# Autodesk Inventor assembly: Assembly.
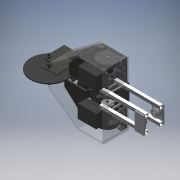
[picture p0: Inventor's stored thumbnail of the model, 180x180]
Saved by Autodesk Inventor 2019 (Build 230136000, 136)
## iProperties
Created: 2018-08-16
Part Number: Assembly.
Document SubType Name: Assembly
Designer: andres2416
Author: andres2416
## Documents named in this file (28)
- O:\Engineering Club Student\Rahul\2018-2019 bot #3\all files\Assembly..iam
- O:\Engineering Club Student\Rahul\2018-2019 bot #3\all files\battery.ipt
- O:\Engineering Club Student\Rahul\2018-2019 bot #3\all files\REAL MOTOR MOUNT 2.75 BOTTOM.ipt
- O:\Engineering Club Student\Rahul\2018-2019 bot #3\all files\REAL MOTOR MOUNT 2.75 TOP.ipt
- O:\Engineering Club Student\Rahul\2018-2019 bot #3\all files\motor.ipt
- O:\Engineering Club Student\Rahul\2018-2019 bot #3\all files\bar for front weapon.ipt
- O:\Engineering Club Student\Rahul\2018-2019 bot #3\all files\standoff.ipt
- O:\Engineering Club Student\Rahul\2018-2019 bot #3\all files\saw blade poly no hole mount.ipt
- O:\Engineering Club Student\Rahul\2018-2019 bot #3\all files\saw blade axle support (hole for arbor).ipt
- O:\Engineering Club Student\Rahul\2018-2019 bot #3\all files\polycarb wall for saw blade.ipt
- O:\Engineering Club Student\Rahul\2018-2019 bot #3\all files\saw blade.ipt
- O:\Engineering Club Student\Rahul\2018-2019 bot #3\all files\6 inch wheel.ipt
- O:\Engineering Club Student\Rahul\2018-2019 bot #3\all files\axle for saw blade.ipt
- O:\Engineering Club Student\Rahul\2018-2019 bot #3\all files\E30-400 motor.ipt
- O:\Engineering Club Student\Rahul\2018-2019 bot #3\all files\MOTOR MOUNT REAL BOTTOM E30 MOTOR.ipt
- O:\Engineering Club Student\Rahul\2018-2019 bot #3\all files\MOTOR MOUNT REAL TOP E3O MOTOR.ipt
- O:\Engineering Club Student\Rahul\2018-2019 bot #3\all files\Very real base.ipt
- O:\Engineering Club Student\Rahul\2018-2019 bot #3\all files\motor mount platform.ipt
- O:\Engineering Club Student\Rahul\2018-2019 bot #3\all files\vex gear.ipt
- O:\Engineering Club Student\Rahul\2018-2019 bot #3\all files\shaft collar for saw blade axle.ipt
- O:\Engineering Club Student\Rahul\2018-2019 bot #3\all files\motor mount platform right side.ipt
- O:\Engineering Club Student\Rahul\2018-2019 bot #3\all files\Front wall.ipt
- O:\Engineering Club Student\Rahul\2018-2019 bot #3\all files\Side wall.ipt
- O:\Engineering Club Student\Rahul\2018-2019 bot #3\all files\rear angled wall.ipt
- O:\Engineering Club Student\Rahul\2018-2019 bot #3\all files\Aluminum Bracket.ipt
- O:\Engineering Club Student\Rahul\2018-2019 bot #3\all files\weapon motor inverted mount.ipt
- O:\Engineering Club Student\Rahul\2018-2019 bot #3\all files\pillowblock].ipt
- O:\Engineering Club Student\Rahul\2018-2019 bot #3\all files\revised pillow block mount.ipt
## Components (59 placed, 27 different names)
1. battery:1 — Mate:10, Flush:20, Flush:21
2. REAL MOTOR MOUNT 2.75 BOTTOM:1 — Insert:8, Insert:39, Insert:40, Flush:15
3. REAL MOTOR MOUNT 2.75 BOTTOM:2 — Insert:37, Insert:38
4. REAL MOTOR MOUNT 2.75 TOP:2 — Insert:11, Insert:12
5. REAL MOTOR MOUNT 2.75 BOTTOM:3 — Insert:11, Insert:12, Insert:31, Insert:32
6. REAL MOTOR MOUNT 2.75 TOP:3 — Insert:13, Insert:14, Mate:1, Flush:39, Flush:40
7. REAL MOTOR MOUNT 2.75 BOTTOM:4 — Insert:7, Insert:13, Insert:14, Insert:29, Insert:30
8. motor:1 — Insert:8, Insert:42, Insert:51
9. motor:2 — Insert:7, Insert:41
10. saw blade poly no hole mount:1 — Mate:14, Flush:27, Flush:28
11. saw blade axle support (hole for arbor):1 — Mate:3, Flush:6, Insert:43
12. polycarb wall for saw blade:1 — Mate:4, Flush:7, Flush:8, Insert:45, Insert:46
13. saw blade:1 — Insert:43, Insert:44
14. 6 inch wheel:1 — Insert:42, Rotation:3
15. 6 inch wheel:2 — Insert:41, Rotation:3
16. axle for saw blade:1 — Insert:44, Insert:47
17. E30-400 motor:1 — Insert:48, Tangent:50, Insert:50, Insert:55
18. MOTOR MOUNT REAL BOTTOM E30 MOTOR:1 — Mate:6, Flush:11, Flush:12, Mate:8, Flush:14
19. MOTOR MOUNT REAL TOP E3O MOTOR:1 — Mate:8, Insert:50, Flush:14
20. MOTOR MOUNT REAL BOTTOM E30 MOTOR:2 — Mate:5, Flush:9, Flush:10, Flush:12, Insert:48, Mate:7, Flush:13
21. MOTOR MOUNT REAL TOP E3O MOTOR:2 — Mate:7, Tangent:50, Flush:13
22. Very real base:1 — Insert:29, Insert:30, Insert:31, Insert:32, Insert:37, Insert:38, Insert:39, Insert:40, Flush:3, Mate:3, Flush:6, Mate:4, Flush:7, Flush:8, Mate:5, Flush:9, Flush:10, Mate:6, Flush:11, Mate:14, Flush:27, Flush:28, Mate:16, Flush:31, Mate:20, Flush:33, Mate:22, Flush:34, Insert:56, Insert:57, Insert:58, Insert:59, Mate:28, Flush:36, Insert:60, Insert:61, Insert:62, Insert:63, Mate:33, Flush:37, Insert:64, Insert:65, Insert:66, Insert:67, Insert:68, Insert:69, Insert:70, Insert:71
23. motor mount platform:1 — Mate:1, Mate:10, Flush:20, Flush:21, Flush:39, Flush:40
24. vex gear:1 — Insert:47
25. vex gear:2 — Insert:55
26. shaft collar for saw blade axle:1 — Insert:45
27. shaft collar for saw blade axle:2 — Insert:46
28. battery:3 — Mate:11, Flush:22
29. REAL MOTOR MOUNT 2.75 TOP:5 — Insert:51, Flush:15, Insert:52, Mate:9, Flush:41
30. REAL MOTOR MOUNT 2.75 TOP:6 — Insert:52, Flush:19
31. motor mount platform right side:1 — Mate:9, Flush:19, Mate:11, Flush:22, Flush:41
32. Side wall:1 — Mate:16, Flush:31, Mate:21, Flush:35, Mate:31, Mate:32
33. rear angled wall:1 — Mate:22, Flush:34, Mate:24, Mate:27
34. rear angled wall:2 — Mate:20, Flush:33, Mate:21, Mate:25, Mate:26
35. Aluminum Bracket:1 — Insert:56, Mate:24
36. Aluminum Bracket:2 — Insert:57, Mate:27
37. Aluminum Bracket:3 — Insert:58, Mate:25
38. Aluminum Bracket:4 — Insert:59, Mate:26
39. Front wall:1 — Mate:28, Flush:35, Flush:36, Mate:29, Mate:30, Mate:34
40. Aluminum Bracket:5 — Insert:61, Mate:30
41. Aluminum Bracket:6 — Insert:60, Mate:29
42. Aluminum Bracket:7 — Insert:65, Mate:36
43. Aluminum Bracket:8 — Insert:64, Mate:35
44. Aluminum Bracket:9 — Insert:63, Mate:32
45. Aluminum Bracket:10 — Insert:62, Mate:31
46. Side wall:2 — Mate:33, Mate:34, Flush:37, Mate:35, Mate:36
47. weapon motor inverted mount:1 — Insert:66, Insert:67
48. pillowblock]:2 — Mate:39, Mate:40, Flush:46
49. bar for front weapon:1 — Insert:78, Insert:79, Mate:38, Flush:44, Flush:45
50. bar for front weapon:2 — Insert:76, Insert:77, Mate:42
51. bar for front weapon:3 — Insert:70, Insert:71, Insert:74, Insert:75, Mate:37, Flush:42, Flush:43
52. bar for front weapon:4 — Insert:68, Insert:69, Insert:72, Insert:73, Mate:40
53. standoff:1 — Insert:75, Insert:78
54. standoff:2 — Insert:74, Insert:79
55. standoff:3 — Insert:73, Insert:76
56. standoff:4 — Insert:72, Insert:77
57. revised pillow block mount:1 — Mate:38, Flush:44, Flush:45, Mate:41, Flush:47
58. revised pillow block mount:2 — Mate:37, Flush:42, Flush:43, Mate:39, Flush:46
59. pillowblock]:3 — Mate:41, Flush:47, Mate:42
## Relationships (118: Insert 50, Mate 34, Flush 32, Tangent 1, RelateRotation 1)
- Insert:7 (-12.7 mm): REAL MOTOR MOUNT 2.75 BOTTOM:4 ↔ motor:2
- Insert:8 (-12.7 mm): REAL MOTOR MOUNT 2.75 BOTTOM:1 ↔ motor:1
- Insert:11: REAL MOTOR MOUNT 2.75 TOP:2 ↔ REAL MOTOR MOUNT 2.75 BOTTOM:3
- Insert:12: REAL MOTOR MOUNT 2.75 TOP:2 ↔ REAL MOTOR MOUNT 2.75 BOTTOM:3
- Insert:13: REAL MOTOR MOUNT 2.75 TOP:3 ↔ REAL MOTOR MOUNT 2.75 BOTTOM:4
- Insert:14: REAL MOTOR MOUNT 2.75 TOP:3 ↔ REAL MOTOR MOUNT 2.75 BOTTOM:4
- Insert:29: REAL MOTOR MOUNT 2.75 BOTTOM:4 ↔ Very real base:1
- Insert:30: REAL MOTOR MOUNT 2.75 BOTTOM:4 ↔ Very real base:1
- Insert:31: REAL MOTOR MOUNT 2.75 BOTTOM:3 ↔ Very real base:1
- Insert:32: REAL MOTOR MOUNT 2.75 BOTTOM:3 ↔ Very real base:1
- Insert:37: REAL MOTOR MOUNT 2.75 BOTTOM:2 ↔ Very real base:1
- Insert:38: REAL MOTOR MOUNT 2.75 BOTTOM:2 ↔ Very real base:1
- Insert:39: REAL MOTOR MOUNT 2.75 BOTTOM:1 ↔ Very real base:1
- Insert:40: REAL MOTOR MOUNT 2.75 BOTTOM:1 ↔ Very real base:1
- Insert:41: motor:2 ↔ 6 inch wheel:2
- Insert:42 (-38.1 mm): motor:1 ↔ 6 inch wheel:1
- Mate:1: REAL MOTOR MOUNT 2.75 TOP:3 ↔ motor mount platform:1
- Flush:3 (12.7 mm): Very real base:1
- Mate:3: saw blade axle support (hole for arbor):1 ↔ Very real base:1
- Flush:6: saw blade axle support (hole for arbor):1 ↔ Very real base:1
- Mate:4: polycarb wall for saw blade:1 ↔ Very real base:1
- Flush:7: polycarb wall for saw blade:1 ↔ Very real base:1
- Flush:8: polycarb wall for saw blade:1 ↔ Very real base:1
- Insert:43 (7.62 mm): saw blade axle support (hole for arbor):1 ↔ saw blade:1
- Insert:44 (-114.3 mm): saw blade:1 ↔ axle for saw blade:1
- Insert:45: polycarb wall for saw blade:1 ↔ shaft collar for saw blade axle:1
- Insert:46: polycarb wall for saw blade:1 ↔ shaft collar for saw blade axle:2
- Insert:47 (-101.6 mm): axle for saw blade:1 ↔ vex gear:1
- Mate:5: MOTOR MOUNT REAL BOTTOM E30 MOTOR:2 ↔ Very real base:1
- Flush:9 (177.8 mm): MOTOR MOUNT REAL BOTTOM E30 MOTOR:2 ↔ Very real base:1
- Flush:10 (165.1 mm): MOTOR MOUNT REAL BOTTOM E30 MOTOR:2 ↔ Very real base:1
- Mate:6: MOTOR MOUNT REAL BOTTOM E30 MOTOR:1 ↔ Very real base:1
- Flush:11 (-241.3 mm): MOTOR MOUNT REAL BOTTOM E30 MOTOR:1 ↔ Very real base:1
- Flush:12: MOTOR MOUNT REAL BOTTOM E30 MOTOR:1 ↔ MOTOR MOUNT REAL BOTTOM E30 MOTOR:2
- Insert:48 (-63.5 mm): E30-400 motor:1 ↔ MOTOR MOUNT REAL BOTTOM E30 MOTOR:2
- Mate:7: MOTOR MOUNT REAL BOTTOM E30 MOTOR:2 ↔ MOTOR MOUNT REAL TOP E3O MOTOR:2
- Tangent:50: E30-400 motor:1 ↔ MOTOR MOUNT REAL TOP E3O MOTOR:2
- Flush:13: MOTOR MOUNT REAL BOTTOM E30 MOTOR:2 ↔ MOTOR MOUNT REAL TOP E3O MOTOR:2
- Mate:8: MOTOR MOUNT REAL BOTTOM E30 MOTOR:1 ↔ MOTOR MOUNT REAL TOP E3O MOTOR:1
- Insert:50: E30-400 motor:1 ↔ MOTOR MOUNT REAL TOP E3O MOTOR:1
- Flush:14: MOTOR MOUNT REAL BOTTOM E30 MOTOR:1 ↔ MOTOR MOUNT REAL TOP E3O MOTOR:1
- Insert:51: motor:1 ↔ REAL MOTOR MOUNT 2.75 TOP:5
- Flush:15: REAL MOTOR MOUNT 2.75 BOTTOM:1 ↔ REAL MOTOR MOUNT 2.75 TOP:5
- Insert:52 (38.1 mm): REAL MOTOR MOUNT 2.75 TOP:5 ↔ REAL MOTOR MOUNT 2.75 TOP:6
- Mate:9: REAL MOTOR MOUNT 2.75 TOP:5 ↔ motor mount platform right side:1
- Flush:19 (-29.21 mm): REAL MOTOR MOUNT 2.75 TOP:6 ↔ motor mount platform right side:1
- Mate:10: battery:1 ↔ motor mount platform:1
- Flush:20 (25.4 mm): battery:1 ↔ motor mount platform:1
- Flush:21: battery:1 ↔ motor mount platform:1
- Mate:11: battery:3 ↔ motor mount platform right side:1
- Flush:22 (25.4 mm): battery:3 ↔ motor mount platform right side:1
- Rotation:3 [RelateRotation] (1 ul): 6 inch wheel:1 ↔ 6 inch wheel:2
- Mate:14: saw blade poly no hole mount:1 ↔ Very real base:1
- Flush:27: saw blade poly no hole mount:1 ↔ Very real base:1
- Flush:28: saw blade poly no hole mount:1 ↔ Very real base:1
- Insert:55 (-34.29 mm): E30-400 motor:1 ↔ vex gear:2
- Mate:16: Very real base:1 ↔ Side wall:1
- Flush:31: Very real base:1 ↔ Side wall:1
- Mate:20: Very real base:1 ↔ rear angled wall:2
- Flush:33: Very real base:1 ↔ rear angled wall:2
- Mate:21: Side wall:1 ↔ rear angled wall:2
- Mate:22: Very real base:1 ↔ rear angled wall:1
- Flush:34: Very real base:1 ↔ rear angled wall:1
- Insert:56: Very real base:1 ↔ Aluminum Bracket:1
- Mate:24: rear angled wall:1 ↔ Aluminum Bracket:1
- Insert:57: Very real base:1 ↔ Aluminum Bracket:2
- Insert:58: Very real base:1 ↔ Aluminum Bracket:3
- Insert:59: Very real base:1 ↔ Aluminum Bracket:4
- Mate:25: rear angled wall:2 ↔ Aluminum Bracket:3
- Mate:26: rear angled wall:2 ↔ Aluminum Bracket:4
- Mate:27: rear angled wall:1 ↔ Aluminum Bracket:2
- Mate:28: Very real base:1 ↔ Front wall:1
- Flush:35: Side wall:1 ↔ Front wall:1
- Flush:36: Very real base:1 ↔ Front wall:1
- Insert:60: Very real base:1 ↔ Aluminum Bracket:6
- Mate:29: Front wall:1 ↔ Aluminum Bracket:6
- Insert:61: Very real base:1 ↔ Aluminum Bracket:5
- Mate:30: Front wall:1 ↔ Aluminum Bracket:5
- Insert:62: Very real base:1 ↔ Aluminum Bracket:10
- Mate:31: Side wall:1 ↔ Aluminum Bracket:10
- Insert:63: Very real base:1 ↔ Aluminum Bracket:9
- Mate:32: Side wall:1 ↔ Aluminum Bracket:9
- Mate:33: Very real base:1 ↔ Side wall:2
- Mate:34: Front wall:1 ↔ Side wall:2
- Flush:37: Very real base:1 ↔ Side wall:2
- Insert:64: Very real base:1 ↔ Aluminum Bracket:8
- Mate:35: Aluminum Bracket:8 ↔ Side wall:2
- Insert:65: Very real base:1 ↔ Aluminum Bracket:7
- Mate:36: Aluminum Bracket:7 ↔ Side wall:2
- Insert:66: Very real base:1 ↔ weapon motor inverted mount:1
- Insert:67: Very real base:1 ↔ weapon motor inverted mount:1
- Insert:68: Very real base:1 ↔ bar for front weapon:4
- Insert:69: Very real base:1 ↔ bar for front weapon:4
- Insert:70: Very real base:1 ↔ bar for front weapon:3
- Insert:71: Very real base:1 ↔ bar for front weapon:3
- Insert:72: bar for front weapon:4 ↔ standoff:4
- Insert:73: bar for front weapon:4 ↔ standoff:3
- Insert:74: bar for front weapon:3 ↔ standoff:2
- Insert:75: bar for front weapon:3 ↔ standoff:1
- Insert:76: bar for front weapon:2 ↔ standoff:3
- Insert:77: bar for front weapon:2 ↔ standoff:4
- Flush:39 (-25.4 mm): REAL MOTOR MOUNT 2.75 TOP:3 ↔ motor mount platform:1
- Flush:40 (-6.35 mm): REAL MOTOR MOUNT 2.75 TOP:3 ↔ motor mount platform:1
- Flush:41: REAL MOTOR MOUNT 2.75 TOP:5 ↔ motor mount platform right side:1
- Insert:78: bar for front weapon:1 ↔ standoff:1
- Insert:79: bar for front weapon:1 ↔ standoff:2
- Mate:37: bar for front weapon:3 ↔ revised pillow block mount:2
- Flush:42: bar for front weapon:3 ↔ revised pillow block mount:2
- Flush:43: bar for front weapon:3 ↔ revised pillow block mount:2
- Mate:38: bar for front weapon:1 ↔ revised pillow block mount:1
- Flush:44: bar for front weapon:1 ↔ revised pillow block mount:1
- Flush:45: bar for front weapon:1 ↔ revised pillow block mount:1
- Mate:39: pillowblock]:2 ↔ revised pillow block mount:2
- Mate:40 (6.35 mm): pillowblock]:2 ↔ bar for front weapon:4
- Flush:46: pillowblock]:2 ↔ revised pillow block mount:2
- Mate:41: revised pillow block mount:1 ↔ pillowblock]:3
- Flush:47: revised pillow block mount:1 ↔ pillowblock]:3
- Mate:42 (6.35 mm): bar for front weapon:2 ↔ pillowblock]:3
